# Autodesk Inventor assembly: Modified EVA Carriage
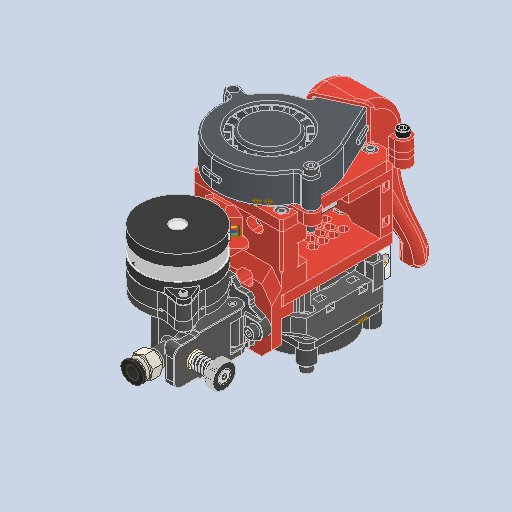
[picture p0: Inventor's stored thumbnail of the model, 512x512]
Saved by Autodesk Inventor 2022 (Build 260153000, 153)
## iProperties
Created: 2021-10-06
Part Number: Modified EVA Carriage
Document SubType Name: Assembly
Designer: Administrator
Title: Modified EVA Carriage v27
Author: Administrator
## Documents named in this file (5)
- Y:\Projects\Bibble0\Modified EVA Carriage\Modified EVA Carriage.iam
- Y:\Projects\Bibble0\Modified EVA Carriage\[Assembly] Orbiter _1_.iam
- Y:\Projects\Bibble0\Modified EVA Carriage\Belt Tensioner.ipt
- Y:\Projects\Bibble0\Modified EVA Carriage\[Face] Dragon v4.iam
- Y:\Projects\Bibble0\Modified EVA Carriage\BL-Touch _1_.iam
## Components (4 placed, 4 different names)
1. [Assembly] Orbiter <1>:1 [sub-assembly] — Insert:2, Mate:1, Flush:1, Mate:2
2. Component94:1 — Mate:1, Flush:1, Mate:2
3. [Face] Dragon v4:1 [sub-assembly] — Insert:1, Insert:2
4. BL Touch v3:1 [sub-assembly] — Insert:1
## Relationships (5: Insert 2, Mate 2, Flush 1)
- Insert:1: [Face] Dragon v4:1 ↔ BL Touch v3:1
- Insert:2: [Assembly] Orbiter <1>:1 ↔ [Face] Dragon v4:1
- Mate:1: [Assembly] Orbiter <1>:1 ↔ Component94:1
- Flush:1: [Assembly] Orbiter <1>:1 ↔ Component94:1
- Mate:2: [Assembly] Orbiter <1>:1 ↔ Component94:1
